# Autodesk Inventor assembly: Finger Assem
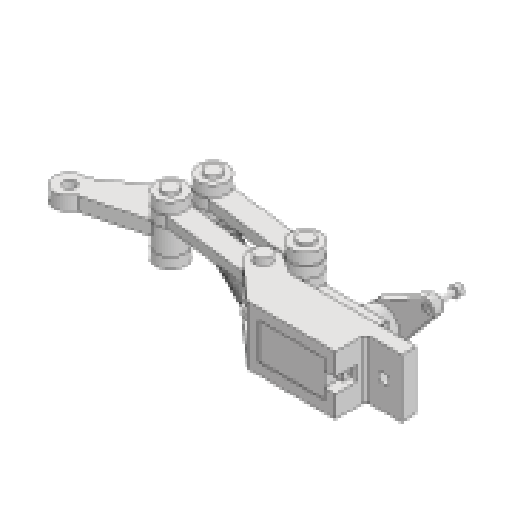
[picture p0: Inventor's stored thumbnail of the model, 512x512]
Saved by Autodesk Inventor 2025.1 (Build 291241020, 241B)
## iProperties
Created: 2024-12-05
Part Number: Finger Assem
Document SubType Name: Assembly
Designer: ALEXANDERNICHOLS
Author: ALEXANDERNICHOLS
## Documents named in this file (13)
- D:\CAD\Inventor\Bio Kettering Hand\Liv Mas 1.0\Finger Assem.iam
- D:\CAD\Inventor\Bio Kettering Hand\Liv Mas 1.0\Arm 1.ipt
- D:\CAD\Inventor\Bio Kettering Hand\Liv Mas 1.0\Arm 2.ipt
- D:\CAD\Inventor\Bio Kettering Hand\Liv Mas 1.0\Arm 3.ipt
- D:\CAD\Inventor\Bio Kettering Hand\Liv Mas 1.0\Servo Base.ipt
- D:\CAD\Inventor\Bio Kettering Hand\Liv Mas 1.0\Servo Spinner.ipt
- D:\CAD\Inventor\Bio Kettering Hand\Liv Mas 1.0\Washer.ipt
- D:\CAD\Inventor\Bio Kettering Hand\Liv Mas 1.0\Servo.ipt
- D:\CAD\Inventor\Bio Kettering Hand\Liv Mas 1.0\Spring Holder.ipt
- D:\CAD\Inventor\Bio Kettering Hand\Liv Mas 1.0\Screw PROP.ipt
- D:\CAD\Inventor\Bio Kettering Hand\Liv Mas 1.0\Spring PROP.ipt
- D:\CAD\Inventor\Bio Kettering Hand\Liv Mas 1.0\Screw BIG 1.ipt
- D:\CAD\Inventor\Bio Kettering Hand\Liv Mas 1.0\Tip Arm 1.ipt
## Components (25 placed, 12 different names)
1. Arm 1:1 — Rotational:2, Rotational:3, Rotational:11, Rotational:14
2. Arm 2:1 — Rotational:11, Rotational:18, Rotational:20, Rotational:30
3. Arm 3:1 — Rotational:1, Rotational:2, Rotational:19
4. Servo Base:1 — Mate:1, Mate:2, Mate:3, Rotational:1, Rotational:24
5. Servo Spinner:1 — Rotational:13, Rotational:25, Rotational:26
6. Washer:1 — Rotational:15
7. Servo:1 — Mate:1, Mate:2, Mate:3, Rotational:13, Rotational:27, Rotational:28
8. Spring Holder:1 — Rotational:16, Mate:5, Rotational:29
9. Spring Holder:2 — Rotational:3, Mate:4, Mate:6
10. Spring Holder:3 — Rotational:14, Rotational:15
11. Washer:2 — Rotational:16
12. Washer:3 — Rotational:31, Mate:7
13. Washer:4 — Rotational:18, Rotational:21
14. Washer:5 — Rotational:19, Rotational:23
15. Washer:6 — Rotational:20, Rotational:22
16. Screw PROP:1 — Rotational:21
17. Screw PROP:2 — Rotational:22
18. Screw PROP:3 — Rotational:23, Mate:7
19. Screw PROP:4 — Rotational:24
20. Spring PROP:1 — Mate:4, Mate:5, Mate:6
21. Screw BIG 1:1 — Rotational:25
22. Screw BIG 1:2 — Rotational:26
23. Screw BIG 1:3 — Rotational:27
24. Screw BIG 1:4 — Rotational:28
25. Tip Arm 1:1 — Rotational:29, Rotational:30, Rotational:31
## Relationships (29: RevoluteJoint 22, Mate 7)
- Mate:1: Servo Base:1 ↔ Servo:1
- Mate:2: Servo Base:1 ↔ Servo:1
- Mate:3: Servo Base:1 ↔ Servo:1
- Rotational:1 [RevoluteJoint]: Arm 3:1 ↔ Servo Base:1
- Rotational:2 [RevoluteJoint]: Arm 1:1 ↔ Arm 3:1
- Rotational:3 [RevoluteJoint]: Arm 1:1 ↔ Spring Holder:2
- Rotational:11 [RevoluteJoint]: Arm 1:1 ↔ Arm 2:1
- Rotational:13 [RevoluteJoint]: Servo Spinner:1 ↔ Servo:1
- Rotational:14 [RevoluteJoint]: Arm 1:1 ↔ Spring Holder:3
- Rotational:15 [RevoluteJoint] (-0.508 mm): Washer:1 ↔ Spring Holder:3
- Rotational:16 [RevoluteJoint] (-0.508 mm): Spring Holder:1 ↔ Washer:2
- Rotational:18 [RevoluteJoint] (0.508 mm): Arm 2:1 ↔ Washer:4
- Rotational:19 [RevoluteJoint] (0.508 mm): Arm 3:1 ↔ Washer:5
- Rotational:20 [RevoluteJoint] (0.508 mm): Arm 2:1 ↔ Washer:6
- Rotational:21 [RevoluteJoint]: Washer:4 ↔ Screw PROP:1
- Rotational:22 [RevoluteJoint]: Washer:6 ↔ Screw PROP:2
- Rotational:23 [RevoluteJoint]: Washer:5 ↔ Screw PROP:3
- Rotational:24 [RevoluteJoint]: Servo Base:1 ↔ Screw PROP:4
- Mate:4: Spring Holder:2 ↔ Spring PROP:1
- Mate:5: Spring Holder:1 ↔ Spring PROP:1
- Mate:6: Spring Holder:2 ↔ Spring PROP:1
- Rotational:25 [RevoluteJoint]: Servo Spinner:1 ↔ Screw BIG 1:1
- Rotational:26 [RevoluteJoint]: Servo Spinner:1 ↔ Screw BIG 1:2
- Rotational:27 [RevoluteJoint]: Servo:1 ↔ Screw BIG 1:3
- Rotational:28 [RevoluteJoint]: Servo:1 ↔ Screw BIG 1:4
- Rotational:29 [RevoluteJoint]: Spring Holder:1 ↔ Tip Arm 1:1
- Rotational:30 [RevoluteJoint]: Arm 2:1 ↔ Tip Arm 1:1
- Rotational:31 [RevoluteJoint]: Washer:3 ↔ Tip Arm 1:1
- Mate:7: Washer:3 ↔ Screw PROP:3
